# Autodesk Inventor assembly: cortex plate
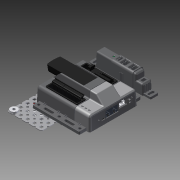
[picture p0: Inventor's stored thumbnail of the model, 180x180]
Saved by Autodesk Inventor 2014 SP1 (Build 180222100, 222)
## iProperties
Created: 2013-10-20
Part Number: cortex plate
Document SubType Name: Assembly
Designer: RyanHughes
Author: RyanHughes
## Documents named in this file (8)
- C:\Users\Ryan\Desktop\sw\toss up 2ed A bot\toss up tower\cortex plate.iam
- C:\Users\Ryan\Desktop\sw\lib\Aperture VEX CAD Library\Metal\Plate\5 x 15.ipt
- C:\Users\Ryan\Desktop\sw\lib\Super Sonic Sparks VEX CAD Library\Other Parts\(VEX) Cortex Microcontroller.iam
- C:\Users\Ryan\Desktop\sw\lib\Super Sonic Sparks VEX CAD Library\Other Parts\Power Expander.iam
- C:\Users\Ryan\Desktop\sw\lib\Super Sonic Sparks VEX CAD Library\Motors & Sensors\Limit Switch (Sensor).iam
- C:\Users\Ryan\Desktop\sw\lib\Aperture VEX CAD Library\Bearing Blocks\Bearing Block.ipt
- C:\Users\Ryan\Desktop\sw\lib\Aperture VEX CAD Library\Spacers\thin\SPACER-0320-0125.ipt
- C:\Users\Ryan\Desktop\sw\lib\Aperture VEX CAD Library\Spacers\SPACER-0500-0125.ipt
## Components (16 placed, 7 different names)
1. 5 x 15:1 — Mate:3, Mate:5, Mate:6, Mate:7, Mate:8, Mate:11, Mate:15, Mate:18, Angle:1, Mate:20, Mate:21, Mate:22, Mate:23, Mate:25, Mate:27, Mate:28, Angle:3, Mate:30, Mate:31, Mate:32, Mate:33, Mate:34, Mate:35, Mate:36
2. (VEX) Cortex Microcontroller:1 [sub-assembly] — Mate:3, Mate:11, Mate:19, Mate:24
3. Power Expander:1 [sub-assembly] — Mate:5, Mate:6, Mate:7, Mate:8
4. SPACER-0500-0125:2 — Mate:15, Mate:21, Mate:22
5. SPACER-0500-0125:3 — Mate:23, Mate:24, Mate:25
6. SPACER-0500-0125:4 — Mate:31, Mate:32, Mate:33
7. SPACER-0500-0125:5 — Mate:34, Mate:35, Mate:36
8. Limit Switch (Sensor):1 [sub-assembly] — Flush:1, Mate:18, Mate:26, Mate:27, Mate:28, Mate:29, Angle:2
9. Bearing Block:1 — Mate:9, Mate:10, Mate:26, Mate:30
10. SPACER-0320-0125:1 — Mate:9, Mate:10, Flush:1
11. Limit Switch (Sensor):2 [sub-assembly]
12. Bearing Block:2
13. SPACER-0320-0125:2
14. Limit Switch (Sensor):3 [sub-assembly]
15. Bearing Block:3
16. SPACER-0320-0125:3
## Component patterns: (3 elements, first: Limit Switch (Sensor):1 + Bearing Block:1 + SPACER-0320-0125:1)
## Relationships (32: Mate 28, Angle 3, Flush 1)
- Mate:3 (2.3114 mm): 5 x 15:1 ↔ (VEX) Cortex Microcontroller:1
- Mate:5: 5 x 15:1 ↔ Power Expander:1
- Mate:6 (-1.0795 mm): 5 x 15:1 ↔ Power Expander:1
- Mate:7 (-1.0795 mm): 5 x 15:1 ↔ Power Expander:1
- Mate:8 (-0.0508 mm): 5 x 15:1 ↔ Power Expander:1
- Mate:9: Bearing Block:1 ↔ SPACER-0320-0125:1
- Mate:10: Bearing Block:1 ↔ SPACER-0320-0125:1
- Flush:1: Limit Switch (Sensor):1 ↔ SPACER-0320-0125:1
- Mate:11 (3.175 mm): 5 x 15:1 ↔ (VEX) Cortex Microcontroller:1
- Mate:15: 5 x 15:1 ↔ SPACER-0500-0125:2
- Mate:18: 5 x 15:1 ↔ Limit Switch (Sensor):1
- Mate:19: (VEX) Cortex Microcontroller:1
- Angle:1 (0 deg): 5 x 15:1
- Mate:20 (-2.54 mm): 5 x 15:1
- Mate:21 (2.3114 mm): 5 x 15:1 ↔ SPACER-0500-0125:2
- Mate:22 (2.3114 mm): 5 x 15:1 ↔ SPACER-0500-0125:2
- Mate:23 (2.3114 mm): 5 x 15:1 ↔ SPACER-0500-0125:3
- Mate:24: (VEX) Cortex Microcontroller:1 ↔ SPACER-0500-0125:3
- Mate:25 (2.3114 mm): 5 x 15:1 ↔ SPACER-0500-0125:3
- Mate:26 (38.1 mm): Limit Switch (Sensor):1 ↔ Bearing Block:1
- Mate:27 (2.3114 mm): 5 x 15:1 ↔ Limit Switch (Sensor):1
- Mate:28 (2.3114 mm): 5 x 15:1 ↔ Limit Switch (Sensor):1
- Mate:29: Limit Switch (Sensor):1
- Angle:2 (90 deg): Limit Switch (Sensor):1
- Angle:3 (180 deg): 5 x 15:1
- Mate:30 (2.3114 mm): 5 x 15:1 ↔ Bearing Block:1
- Mate:31: 5 x 15:1 ↔ SPACER-0500-0125:4
- Mate:32 (2.3114 mm): 5 x 15:1 ↔ SPACER-0500-0125:4
- Mate:33 (2.3114 mm): 5 x 15:1 ↔ SPACER-0500-0125:4
- Mate:34: 5 x 15:1 ↔ SPACER-0500-0125:5
- Mate:35 (2.3114 mm): 5 x 15:1 ↔ SPACER-0500-0125:5
- Mate:36 (2.3114 mm): 5 x 15:1 ↔ SPACER-0500-0125:5
## Named parameters: q = 2.3114 mm
